# Autodesk Inventor assembly: single_wheel_dummie
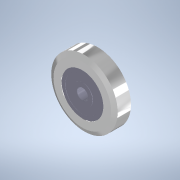
[picture p0: Inventor's stored thumbnail of the model, 180x180]
Saved by Autodesk Inventor 2020.3 (Build 243373000, 373)
## iProperties
Created: 2021-03-25
Part Number: single_wheel_dummie
Document SubType Name: Assembly
Designer: patry
Author: patry
## Documents named in this file (3)
- C:\Users\patry\Desktop\Konar staff\Ariadna2.1\ariadna_mechanika\Obszar roboczy\Naped\Kola\single_wheel_dummie.iam
- C:\Users\patry\Desktop\Konar staff\Ariadna2.1\ariadna_mechanika\Obszar roboczy\Naped\Lozyska\6352RS-5mm\635-2RS-TheTimkenCompany-3D-03-22-2021.ipt
- C:\Users\patry\Desktop\Konar staff\Ariadna2.1\ariadna_mechanika\Obszar roboczy\Naped\Kola\opona_nosne_dummie.ipt
## Components (2 placed, 2 different names)
1. 635-2RS-TheTimkenCompany-3D-03-22-2021:1 — Zestawiające:1, Zestawiające:2
2. opona_nosne_dummie:1 — Zestawiające:1, Zestawiające:2
## Relationships (2: Mate 2)
- Zestawiające:1 [Mate]: 635-2RS-TheTimkenCompany-3D-03-22-2021:1 ↔ opona_nosne_dummie:1
- Zestawiające:2 [Mate]: 635-2RS-TheTimkenCompany-3D-03-22-2021:1 ↔ opona_nosne_dummie:1
